# Autodesk Inventor assembly: YZ_GANTRY
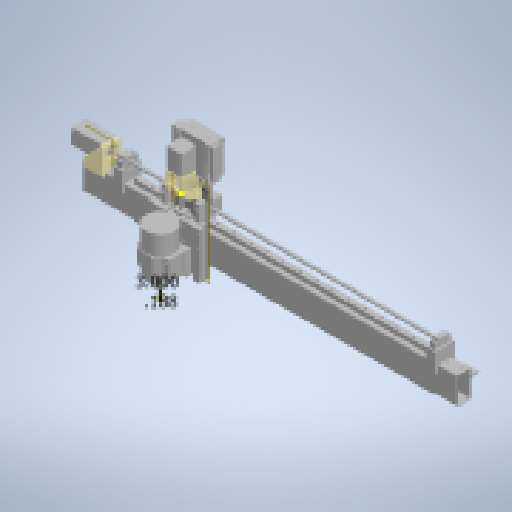
[picture p0: Inventor's stored thumbnail of the model, 512x512]
Saved by Autodesk Inventor 2023 (Build 270158000, 158)
## iProperties
Created: 2023-06-21
Part Number: YZ_GANTRY
Document SubType Name: Assembly
Designer: plebbb
Author: plebbb
## Documents named in this file (5)
- G:\CNC PROJECT\CNC_Project\YZ_GANTRY.iam
- G:\CNC PROJECT\CNC_Project\Z_GANTRY.iam
- G:\CNC PROJECT\CNC_Project\Y_GANTRY.iam
- G:\CNC PROJECT\CNC_Project\Cable_Chain_Side_Holder.ipt
- G:\CNC PROJECT\CNC_Project\Cable_Chain_Holder_Gantry.ipt
## Components (4 placed, 4 different names)
1. Z_GANTRY:1 [sub-assembly] — Flush:2
2. Y_GANTRY:1 [sub-assembly] — Mate:27
3. Cable_Chain_Side_Holder:1 — Mate:27
4. Cable_Chain_Holder_Gantry:1 — Flush:2
## Relationships (11: Mate 9, Flush 2)
- [Mate]: Z_GANTRY:1 ↔ Y_GANTRY:1
- [Mate]: Z_GANTRY:1 ↔ Y_GANTRY:1
- [Mate]: Z_GANTRY:1 ↔ Y_GANTRY:1
- [Mate]: Z_GANTRY:1 ↔ Y_GANTRY:1
- [Mate]: Z_GANTRY:1 ↔ Y_GANTRY:1
- [Mate]: Z_GANTRY:1 ↔ Y_GANTRY:1
- [Mate]: Z_GANTRY:1 ↔ Y_GANTRY:1
- [Mate]: Y_GANTRY:1 ↔ Cable_Chain_Side_Holder:1
- [Flush] (45 mm): Y_GANTRY:1 ↔ Cable_Chain_Side_Holder:1
- Mate:27 (-30 mm): Y_GANTRY:1 ↔ Cable_Chain_Side_Holder:1
- Flush:2: Z_GANTRY:1 ↔ Cable_Chain_Holder_Gantry:1
## Named parameters: d32_d65 = 0 mm, d33_d66 = 0 mm
